# Autodesk Inventor assembly: BASE
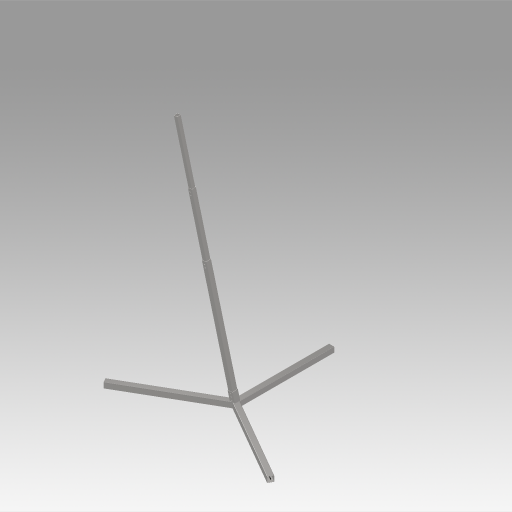
[picture p0: Inventor's stored thumbnail of the model, 512x512]
Saved by Autodesk Inventor 2023 (Build 270158000, 158)
## iProperties
_SolveAssemblyDoc: Frame Generator Solve Assembly
_Version: 25.0.0
Created: 2025-03-27
Part Number: BASE
Document SubType Name: Assembly
Designer: NELLY NDUNG'U
Mass: 67680.8 g
Surface Area: 57485.5 cm^2
Volume: 8621.75 cm^3
Density: 7.85 g/cm^3
Author: NELLY NDUNG'U
## Documents named in this file (15)
- N:\NAKUJA\CAD FILES\AIRFRAME\LP001\BASE.iam
- N:\NAKUJA\CAD FILES\AIRFRAME\LP001\BASE.ipt
- N:\NAKUJA\CAD FILES\AIRFRAME\LP001\BASE\Frame\Frame 1743054956771.iam
- N:\NAKUJA\CAD FILES\AIRFRAME\LP001\LP01.iam
- N:\NAKUJA\CAD FILES\AIRFRAME\LP001\LP02.iam
- N:\NAKUJA\CAD FILES\AIRFRAME\LP001\LP02_2.iam
- C:\Users\User\Documents\Inventor\Content Center Files\R2023\en-US\ANSI B18.2.3.5M\ANSI B18.2.3.5M - M10 x 1.5 x 100.ipt
- C:\Users\User\Documents\Inventor\Content Center Files\R2023\en-US\ANSI B 18.2.4.1 M(1)\ANSI B 18.2.4.1 M - M10 x 1.5Style 1.ipt
- C:\Users\User\Documents\Inventor\Content Center Files\R2023\en-US\ANSI B18.2.3.5M\ANSI B18.2.3.5M - M10 x 1.5 x 90.ipt
- N:\NAKUJA\CAD FILES\AIRFRAME\LP001\BASE\AIP\FEA\f0uqydhfk.fins
- N:\NAKUJA\CAD FILES\AIRFRAME\LP001\BASE\AIP\FEA\f0uqydhfk.fsat
- N:\NAKUJA\CAD FILES\AIRFRAME\LP001\BASE\AIP\FEA\f0uqydhfk.ftes
- N:\NAKUJA\CAD FILES\AIRFRAME\LP001\BASE\AIP\FEA\f0uqydhfk.fwiz
- N:\NAKUJA\CAD FILES\AIRFRAME\LP001\BASE\AIP\FEA\f0uqydhk0.fmsh
- N:\NAKUJA\CAD FILES\AIRFRAME\LP001\BASE\AIP\FEA\f0uqydhkw.fres
## Components (19 placed, 8 different names)
1. BASE:1
2. Frame 1743054956771:1 [sub-assembly] — Mate:11, Mate:12, Mate:13, Insert:1, Insert:2, Insert:3, Insert:4, Insert:5, Insert:6
3. LP01:1 [sub-assembly] — Mate:5, Mate:6, Mate:7, Mate:11, Mate:12, Mate:13, Insert:7, Insert:8, Insert:9, Insert:10
4. LP02:1 [sub-assembly] — Mate:5, Mate:6, Mate:7, Mate:8, Mate:9, Mate:10, Insert:11, Insert:12, Insert:13, Insert:14
5. LP02_2:1 [sub-assembly] — Mate:8, Mate:9, Mate:10
6. Hex Bolt - Metric M10 x 1.5 x 100:1 — Insert:3
7. Hex Bolt - Metric M10 x 1.5 x 100:2 — Insert:2
8. Hex Bolt - Metric M10 x 1.5 x 100:3 — Insert:1
9. Hex Nut Metric M10 x 1.5:1 — Insert:6
10. Hex Nut Metric M10 x 1.5:2 — Insert:4
11. Hex Nut Metric M10 x 1.5:3 — Insert:5
12. Hex Bolt - Metric M10 x 1.5 x 100:4 — Insert:7
13. Hex Bolt - Metric M10 x 1.5 x 100:5 — Insert:8
14. Hex Nut Metric M10 x 1.5:4 — Insert:9
15. Hex Nut Metric M10 x 1.5:5 — Insert:10
16. Hex Bolt - Metric M10 x 1.5 x 90:1 — Insert:11
17. Hex Bolt - Metric M10 x 1.5 x 90:2 — Insert:12
18. Hex Nut Metric M10 x 1.5:6 — Insert:13
19. Hex Nut Metric M10 x 1.5:7 — Insert:14
## Relationships (23: Insert 14, Mate 9)
- Mate:5 (2 mm): LP01:1 ↔ LP02:1
- Mate:6 (2 mm): LP01:1 ↔ LP02:1
- Mate:7 (-125 mm): LP01:1 ↔ LP02:1
- Mate:8 (2 mm): LP02:1 ↔ LP02_2:1
- Mate:9 (2 mm): LP02:1 ↔ LP02_2:1
- Mate:10 (-125 mm): LP02:1 ↔ LP02_2:1
- Mate:11 (2 mm): Frame 1743054956771:1 ↔ LP01:1
- Mate:12 (2 mm): Frame 1743054956771:1 ↔ LP01:1
- Mate:13 (-151.195 mm): Frame 1743054956771:1 ↔ LP01:1
- Insert:1: Frame 1743054956771:1 ↔ Hex Bolt - Metric M10 x 1.5 x 100:3
- Insert:2: Frame 1743054956771:1 ↔ Hex Bolt - Metric M10 x 1.5 x 100:2
- Insert:3: Frame 1743054956771:1 ↔ Hex Bolt - Metric M10 x 1.5 x 100:1
- Insert:4: Frame 1743054956771:1 ↔ Hex Nut Metric M10 x 1.5:2
- Insert:5: Frame 1743054956771:1 ↔ Hex Nut Metric M10 x 1.5:3
- Insert:6: Frame 1743054956771:1 ↔ Hex Nut Metric M10 x 1.5:1
- Insert:7: LP01:1 ↔ Hex Bolt - Metric M10 x 1.5 x 100:4
- Insert:8: LP01:1 ↔ Hex Bolt - Metric M10 x 1.5 x 100:5
- Insert:9: LP01:1 ↔ Hex Nut Metric M10 x 1.5:4
- Insert:10: LP01:1 ↔ Hex Nut Metric M10 x 1.5:5
- Insert:11: LP02:1 ↔ Hex Bolt - Metric M10 x 1.5 x 90:1
- Insert:12: LP02:1 ↔ Hex Bolt - Metric M10 x 1.5 x 90:2
- Insert:13: LP02:1 ↔ Hex Nut Metric M10 x 1.5:6
- Insert:14: LP02:1 ↔ Hex Nut Metric M10 x 1.5:7
## Named parameters: sa_0 = 104200
note: some values were not read from the file. Shown as the stored number, unit unknown: "sa_0".
